# Autodesk Inventor assembly: 000.005.001 - Поворотный стол
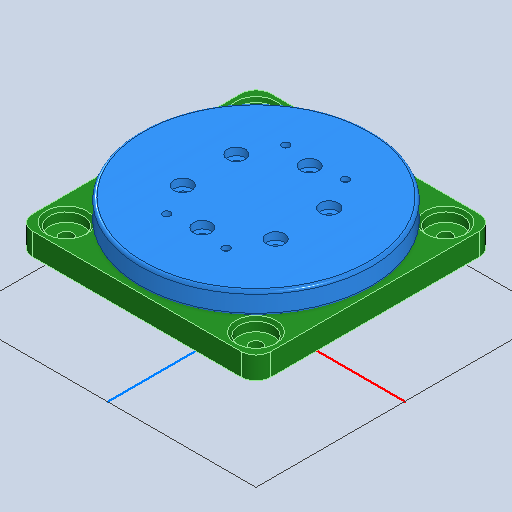
[picture p0: Inventor's stored thumbnail of the model, 512x512]
Saved by Autodesk Inventor 2022 (Build 260153000, 153)
## iProperties
Created: 2022-11-17
Part Number: 000.005.001 - Поворотный стол
Document SubType Name: Assembly
Designer: Petrov Ivan
Author: Petrov Ivan
## Documents named in this file (11)
- D:\IVAN\Ivan_desktop\Kvantorium\Projects\YouBotRobot\design\000.005.001 - Поворотный стол.iam
- D:\IVAN\Ivan_desktop\Kvantorium\Projects\YouBotRobot\design\000.005.001.001 - Основание.ipt
- D:\IVAN\Ivan_desktop\Kvantorium\Projects\YouBotRobot\design\000.005.001.002 - Шар.ipt
- D:\IVAN\Ivan_desktop\Kvantorium\Projects\YouBotRobot\design\000.005.001.002 - Поворотное основание.ipt
- D:\IVAN\Ivan_desktop\Kvantorium\Projects\YouBotRobot\design\000.005.001.003 - Вал.ipt
- D:\IVAN\Ivan_desktop\Kvantorium\Projects\YouBotRobot\design\standart_components\dynamixels\mx-64\MX-64T.iam
- D:\IVAN\Ivan_desktop\Kvantorium\Projects\YouBotRobot\design\Content Center Files\R2022\ru-RU\BS EN 24035\ISO 4035 - M5BS EN.ipt
- C:\Users\Petrov Ivan\Documents\Inventor\Content Center Files\R2022\ru-RU\ISO 4762(1)\DIN EN ISO 4762 - M5 x 10.ipt
- C:\Users\Petrov Ivan\Documents\Inventor\Content Center Files\R2022\ru-RU\IS 2269\IS 2269 - M2,5 x 10.ipt
- C:\Users\Petrov Ivan\Documents\Inventor\Content Center Files\R2022\ru-RU\BS EN 24 036\BS EN 24 036 - M2.5.ipt
- C:\Users\Petrov Ivan\Documents\Inventor\Content Center Files\R2022\ru-RU\BS EN 24034\ISO 4034 - M5BS EN.ipt
## Components (81 placed, 10 different names)
1. 000.005.001.001 - Основание:1 — Касательность:1, Совмещение:2, Совмещение:3, Совмещение:4, Угол:1, Совмещение:5, Совмещение:8, Совмещение:9, Совмещение:13, Вставка:30, Вставка:31, Вставка:32, Вставка:33, Вставка:34, Вставка:35, Вставка:36, Вставка:37
2. 000.005.001.002 - Поворотное основание:1 — Совмещение:4, Угол:1, Совмещение:5, Совмещение:7, Совмещение:10, Совмещение:11, Вставка:7, Вставка:8, Вставка:9, Вставка:10, Вставка:11, Вставка:12, Вставка:13, Вставка:38, Вставка:39, Вставка:40, Вставка:41
3. 000.005.001.003 - Вал:1 — Совмещение:7, Совмещение:10, Совмещение:11, Совмещение:12, Вставка:1, Вставка:2, Вставка:3, Вставка:4, Вставка:5, Вставка:6, Вставка:14, Вставка:15, Вставка:16, Вставка:17, Вставка:18, Вставка:19, Вставка:20, Вставка:21
4. MX-64T:1 [sub-assembly] — Совмещение:8, Совмещение:9, Совмещение:12, Совмещение:13, Вставка:22, Вставка:23, Вставка:24, Вставка:25, Вставка:26, Вставка:27, Вставка:28, Вставка:29
5. BS EN 24034 - метрическая M5:1 — Вставка:38
6. BS EN 24034 - метрическая M5:2 — Вставка:39
7. BS EN 24034 - метрическая M5:3 — Вставка:40
8. BS EN 24034 - метрическая M5:4 — Вставка:41
9. DIN EN ISO 4762 M5 x 10:1 — Вставка:7
10. DIN EN ISO 4762 M5 x 10:2 — Вставка:8
11. DIN EN ISO 4762 M5 x 10:3 — Вставка:9
12. DIN EN ISO 4762 M5 x 10:4 — Вставка:10
13. DIN EN ISO 4762 M5 x 10:5 — Вставка:11
14. DIN EN ISO 4762 M5 x 10:6 — Вставка:12
15. DIN EN ISO 4762 M5 x 10:7 — Вставка:13
16. BS EN 24035 - метрическая M5:1 — Вставка:1
17. BS EN 24035 - метрическая M5:2 — Вставка:2
18. BS EN 24035 - метрическая M5:3 — Вставка:3
19. BS EN 24035 - метрическая M5:4 — Вставка:4
20. BS EN 24035 - метрическая M5:5 — Вставка:5
21. BS EN 24035 - метрическая M5:6 — Вставка:6
22. IS 2269 M2,5 x 10:9 — Вставка:30
23. IS 2269 M2,5 x 10:10 — Вставка:31
24. IS 2269 M2,5 x 10:11 — Вставка:32
25. IS 2269 M2,5 x 10:12 — Вставка:33
26. IS 2269 M2,5 x 10:13 — Вставка:34
27. IS 2269 M2,5 x 10:14 — Вставка:35
28. IS 2269 M2,5 x 10:15 — Вставка:36
29. IS 2269 M2,5 x 10:16 — Вставка:37
30. IS 2269 M2,5 x 10:1 — Вставка:14
31. IS 2269 M2,5 x 10:2 — Вставка:15
32. IS 2269 M2,5 x 10:3 — Вставка:16
33. IS 2269 M2,5 x 10:4 — Вставка:17
34. IS 2269 M2,5 x 10:5 — Вставка:18
35. IS 2269 M2,5 x 10:6 — Вставка:19
36. IS 2269 M2,5 x 10:7 — Вставка:20
37. IS 2269 M2,5 x 10:8 — Вставка:21
38. BS EN 24036 M2.5:1 — Вставка:22
39. BS EN 24036 M2.5:2 — Вставка:23
40. BS EN 24036 M2.5:3 — Вставка:24
41. BS EN 24036 M2.5:4 — Вставка:25
42. BS EN 24036 M2.5:5 — Вставка:26
43. BS EN 24036 M2.5:6 — Вставка:27
44. BS EN 24036 M2.5:7 — Вставка:28
45. BS EN 24036 M2.5:8 — Вставка:29
46. 000.005.001.002 - Шар:1 — Касательность:1, Совмещение:1
47. 000.005.001.002 - Шар:2
48. 000.005.001.002 - Шар:3
49. 000.005.001.002 - Шар:4
50. 000.005.001.002 - Шар:5
51. 000.005.001.002 - Шар:6
52. 000.005.001.002 - Шар:7
53. 000.005.001.002 - Шар:8
54. 000.005.001.002 - Шар:9
55. 000.005.001.002 - Шар:10
56. 000.005.001.002 - Шар:11
57. 000.005.001.002 - Шар:12
58. 000.005.001.002 - Шар:13
59. 000.005.001.002 - Шар:14
60. 000.005.001.002 - Шар:15
61. 000.005.001.002 - Шар:16
62. 000.005.001.002 - Шар:17
63. 000.005.001.002 - Шар:18
64. 000.005.001.002 - Шар:19
65. 000.005.001.002 - Шар:20
66. 000.005.001.002 - Шар:21
67. 000.005.001.002 - Шар:22
68. 000.005.001.002 - Шар:23
69. 000.005.001.002 - Шар:24
70. 000.005.001.002 - Шар:25
71. 000.005.001.002 - Шар:26
72. 000.005.001.002 - Шар:27
73. 000.005.001.002 - Шар:28
74. 000.005.001.002 - Шар:29
75. 000.005.001.002 - Шар:30
76. 000.005.001.002 - Шар:31
77. 000.005.001.002 - Шар:32
78. 000.005.001.002 - Шар:33
79. 000.005.001.002 - Шар:34
80. 000.005.001.002 - Шар:35
81. 000.005.001.002 - Шар:36
## Component patterns: (36 elements, first: 000.005.001.002 - Шар:1)
## Relationships (55: Insert 41, Mate 12, Tangent 1, Angle 1)
- Касательность:1 [Tangent]: 000.005.001.001 - Основание:1 ↔ 000.005.001.002 - Шар:1
- Совмещение:1 [Mate]: 000.005.001.002 - Шар:1
- Совмещение:2 [Mate]: 000.005.001.001 - Основание:1
- Совмещение:3 [Mate]: 000.005.001.001 - Основание:1
- Совмещение:4 [Mate]: 000.005.001.001 - Основание:1 ↔ 000.005.001.002 - Поворотное основание:1
- Угол:1 [Angle] (180 deg): 000.005.001.001 - Основание:1 ↔ 000.005.001.002 - Поворотное основание:1
- Совмещение:5 [Mate]: 000.005.001.001 - Основание:1 ↔ 000.005.001.002 - Поворотное основание:1
- Совмещение:7 [Mate]: 000.005.001.002 - Поворотное основание:1 ↔ 000.005.001.003 - Вал:1
- Совмещение:8 [Mate]: 000.005.001.001 - Основание:1 ↔ MX-64T:1
- Совмещение:9 [Mate]: 000.005.001.001 - Основание:1 ↔ MX-64T:1
- Совмещение:10 [Mate]: 000.005.001.002 - Поворотное основание:1 ↔ 000.005.001.003 - Вал:1
- Совмещение:11 [Mate]: 000.005.001.002 - Поворотное основание:1 ↔ 000.005.001.003 - Вал:1
- Совмещение:12 [Mate]: 000.005.001.003 - Вал:1 ↔ MX-64T:1
- Совмещение:13 [Mate]: 000.005.001.001 - Основание:1 ↔ MX-64T:1
- Вставка:1 [Insert]: 000.005.001.003 - Вал:1 ↔ BS EN 24035 - метрическая M5:1
- Вставка:2 [Insert]: 000.005.001.003 - Вал:1 ↔ BS EN 24035 - метрическая M5:2
- Вставка:3 [Insert]: 000.005.001.003 - Вал:1 ↔ BS EN 24035 - метрическая M5:3
- Вставка:4 [Insert]: 000.005.001.003 - Вал:1 ↔ BS EN 24035 - метрическая M5:4
- Вставка:5 [Insert]: 000.005.001.003 - Вал:1 ↔ BS EN 24035 - метрическая M5:5
- Вставка:6 [Insert]: 000.005.001.003 - Вал:1 ↔ BS EN 24035 - метрическая M5:6
- Вставка:7 [Insert]: 000.005.001.002 - Поворотное основание:1 ↔ DIN EN ISO 4762 M5 x 10:1
- Вставка:8 [Insert]: 000.005.001.002 - Поворотное основание:1 ↔ DIN EN ISO 4762 M5 x 10:2
- Вставка:9 [Insert]: 000.005.001.002 - Поворотное основание:1 ↔ DIN EN ISO 4762 M5 x 10:3
- Вставка:10 [Insert]: 000.005.001.002 - Поворотное основание:1 ↔ DIN EN ISO 4762 M5 x 10:4
- Вставка:11 [Insert]: 000.005.001.002 - Поворотное основание:1 ↔ DIN EN ISO 4762 M5 x 10:5
- Вставка:12 [Insert]: 000.005.001.002 - Поворотное основание:1 ↔ DIN EN ISO 4762 M5 x 10:6
- Вставка:13 [Insert]: 000.005.001.002 - Поворотное основание:1 ↔ DIN EN ISO 4762 M5 x 10:7
- Вставка:14 [Insert]: 000.005.001.003 - Вал:1 ↔ IS 2269 M2,5 x 10:1
- Вставка:15 [Insert]: 000.005.001.003 - Вал:1 ↔ IS 2269 M2,5 x 10:2
- Вставка:16 [Insert]: 000.005.001.003 - Вал:1 ↔ IS 2269 M2,5 x 10:3
- Вставка:17 [Insert]: 000.005.001.003 - Вал:1 ↔ IS 2269 M2,5 x 10:4
- Вставка:18 [Insert]: 000.005.001.003 - Вал:1 ↔ IS 2269 M2,5 x 10:5
- Вставка:19 [Insert]: 000.005.001.003 - Вал:1 ↔ IS 2269 M2,5 x 10:6
- Вставка:20 [Insert]: 000.005.001.003 - Вал:1 ↔ IS 2269 M2,5 x 10:7
- Вставка:21 [Insert]: 000.005.001.003 - Вал:1 ↔ IS 2269 M2,5 x 10:8
- Вставка:22 [Insert]: MX-64T:1 ↔ BS EN 24036 M2.5:1
- Вставка:23 [Insert]: MX-64T:1 ↔ BS EN 24036 M2.5:2
- Вставка:24 [Insert]: MX-64T:1 ↔ BS EN 24036 M2.5:3
- Вставка:25 [Insert]: MX-64T:1 ↔ BS EN 24036 M2.5:4
- Вставка:26 [Insert]: MX-64T:1 ↔ BS EN 24036 M2.5:5
- Вставка:27 [Insert]: MX-64T:1 ↔ BS EN 24036 M2.5:6
- Вставка:28 [Insert]: MX-64T:1 ↔ BS EN 24036 M2.5:7
- Вставка:29 [Insert]: MX-64T:1 ↔ BS EN 24036 M2.5:8
- Вставка:30 [Insert]: 000.005.001.001 - Основание:1 ↔ IS 2269 M2,5 x 10:9
- Вставка:31 [Insert]: 000.005.001.001 - Основание:1 ↔ IS 2269 M2,5 x 10:10
- Вставка:32 [Insert]: 000.005.001.001 - Основание:1 ↔ IS 2269 M2,5 x 10:11
- Вставка:33 [Insert]: 000.005.001.001 - Основание:1 ↔ IS 2269 M2,5 x 10:12
- Вставка:34 [Insert]: 000.005.001.001 - Основание:1 ↔ IS 2269 M2,5 x 10:13
- Вставка:35 [Insert]: 000.005.001.001 - Основание:1 ↔ IS 2269 M2,5 x 10:14
- Вставка:36 [Insert]: 000.005.001.001 - Основание:1 ↔ IS 2269 M2,5 x 10:15
- Вставка:37 [Insert]: 000.005.001.001 - Основание:1 ↔ IS 2269 M2,5 x 10:16
- Вставка:38 [Insert]: 000.005.001.002 - Поворотное основание:1 ↔ BS EN 24034 - метрическая M5:1
- Вставка:39 [Insert]: 000.005.001.002 - Поворотное основание:1 ↔ BS EN 24034 - метрическая M5:2
- Вставка:40 [Insert]: 000.005.001.002 - Поворотное основание:1 ↔ BS EN 24034 - метрическая M5:3
- Вставка:41 [Insert]: 000.005.001.002 - Поворотное основание:1 ↔ BS EN 24034 - метрическая M5:4
